# Autodesk Inventor assembly: 15102898-16-A-0500
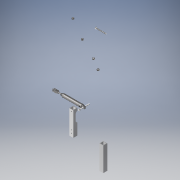
[picture p0: Inventor's stored thumbnail of the model, 180x180]
Saved by Autodesk Inventor 2017 (Build 210142000, 142)
## iProperties
Created: 2016-10-08
Part Number: 15102898-16-A-0500
Document SubType Name: Assembly
Designer: 15102898
Author: 15102898
## Documents named in this file (10)
- C:\Users\15102898\Documents\GitHub\bps-bunnybots2016-cad\Bunnybot-To_be_renamed\15102898-16-A-0000\15102898-16-A-0500.iam
- C:\Users\15102898\Documents\GitHub\bps-bunnybots2016-cad\Bunnybot-To_be_renamed\15102898-16-A-0000\15102898-16-A-0500\15102898-16-A-0501.iam
- C:\Users\15102898\Documents\GitHub\bps-bunnybots2016-cad\Bunnybot-To_be_renamed\15102898-16-A-0000\15102898-16-A-0500\15102898-16-A-0502.iam
- C:\Users\15102898\Documents\GitHub\bps-bunnybots2016-cad\Bunnybot-To_be_renamed\15102898-16-A-0000\15102898-16-A-0500\15102898-16-P-0500.ipt
- C:\Users\15102898\Documents\GitHub\bps-bunnybots2016-cad\Bunnybot-To_be_renamed\15102898-16-A-0000\15102898-16-A-0500\15102898-16-P-0501.ipt
- C:\Users\15102898\Documents\GitHub\bps-bunnybots2016-cad\Bunnybot-To_be_renamed\15102898-16-A-0000\15102898-16-A-0500\15102898-16-P-0503.ipt
- C:\Users\15102898\Documents\GitHub\bps-bunnybots2016-cad\Bunnybot-To_be_renamed\15102898-16-A-0000\15102898-16-P-0505.ipt
- C:\Users\15102898\Documents\GitHub\bps-bunnybots2016-cad\Bunnybot-To_be_renamed\15102898-16-A-0000\15102898-16-A-0500\15102898-16-P-0505.ipt
- C:\Users\15102898\Documents\GitHub\bps-bunnybots2016-cad\Bunnybot-To_be_renamed\15102898-16-A-0000\15102898-16-A-0500\15102898-16-P-0506.ipt
- C:\Users\15102898\Documents\GitHub\bps-bunnybots2016-cad\Bunnybot-To_be_renamed\15102898-16-A-0000\15102898-16-A-0500\15102898-16-P-0508.ipt
## Components (16 placed, 8 different names)
1. 15102898-16-A-0501:1 [sub-assembly] — Cylindrical:1, Mate:1, Mate:3, Mate:4
2. 15102898-16-A-0502:1 [sub-assembly] — Cylindrical:1, Cylindrical:2
3. 15102898-16-P-0500:1 — Mate:2, Mate:3
4. 15102898-16-P-0500:2
5. 15102898-16-P-0500:3
6. 15102898-16-P-0500:4
7. 15102898-16-P-0501:1
8. 15102898-16-P-0503:1
9. 15102898-16-P-0503:2
10. 15102898-16-P-0505:1 — Cylindrical:2, Mate:5, Mate:6
11. 15102898-16-P-0505:2
12. 15102898-16-P-0505:3 — Mate:1, Mate:2, Mate:4
13. 15102898-16-P-0506:1
14. 15102898-16-P-0506:2
15. 15102898-16-P-0508:1
16. 15102898-16-P-0508:2 — Mate:5, Mate:6
## Relationships (8: Mate 6, CylindricalJoint 2)
- Cylindrical:1: 15102898-16-A-0501:1 ↔ 15102898-16-A-0502:1
- Mate:1: 15102898-16-A-0501:1 ↔ 15102898-16-P-0505:3
- Mate:2: 15102898-16-P-0500:1 ↔ 15102898-16-P-0505:3
- Mate:3: 15102898-16-A-0501:1 ↔ 15102898-16-P-0500:1
- Mate:4: 15102898-16-A-0501:1 ↔ 15102898-16-P-0505:3
- Cylindrical:2: 15102898-16-A-0502:1 ↔ 15102898-16-P-0505:1
- Mate:5: 15102898-16-P-0505:1 ↔ 15102898-16-P-0508:2
- Mate:6: 15102898-16-P-0505:1 ↔ 15102898-16-P-0508:2
